# Autodesk Inventor assembly: Section 1
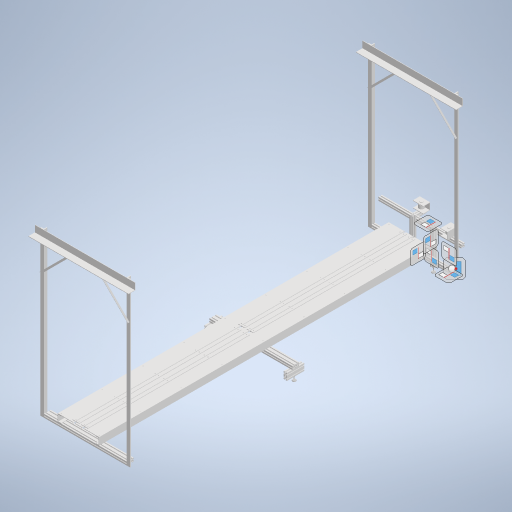
[picture p0: Inventor's stored thumbnail of the model, 512x512]
Saved by Autodesk Inventor 2023 (Build 270158030, 158C)
## iProperties
Created: 2022-06-28
Part Number: Section 1
Document SubType Name: Assembly
Designer: jeremyy
Author: jeremyy
## Documents named in this file (16)
- \\andrew.ad.cmu.edu\users\users1\jeremyy\Documents\Inventor\CMU Bridge\New folder\Section 1.iam
- \\andrew.ad.cmu.edu\users\users1\jeremyy\Documents\Inventor\CMU Bridge\New folder\LatX24in.ipt
- \\andrew.ad.cmu.edu\users\users1\jeremyy\Documents\Inventor\CMU Bridge\New folder\VertL46in.ipt
- \\andrew.ad.cmu.edu\users\users1\jeremyy\Documents\Inventor\CMU Bridge\New folder\LatL29in.ipt
- \\andrew.ad.cmu.edu\users\users1\jeremyy\Documents\Inventor\CMU Bridge\New folder\DiagL.ipt
- \\andrew.ad.cmu.edu\users\users1\jeremyy\Documents\Inventor\CMU Bridge\New folder\DiagR.ipt
- \\andrew.ad.cmu.edu\users\users1\jeremyy\Documents\Inventor\CMU Bridge\New folder\LongC96.ipt
- \\andrew.ad.cmu.edu\users\users1\jeremyy\Documents\Inventor\CMU Bridge\New folder\LatXX24in.ipt
- \\andrew.ad.cmu.edu\users\users1\jeremyy\Documents\Inventor\CMU Bridge\New folder\VertL47.25in.ipt
- \\andrew.ad.cmu.edu\users\users1\jeremyy\Documents\Inventor\CMU Bridge\New folder\LongXX5.ipt
- \\andrew.ad.cmu.edu\users\users1\jeremyy\Documents\Inventor\CMU Bridge\New folder\VertX10EndFoot.ipt
- \\andrew.ad.cmu.edu\users\users1\jeremyy\Documents\Inventor\CMU Bridge\New folder\Foot.ipt
- \\andrew.ad.cmu.edu\users\users1\jeremyy\Documents\Inventor\CMU Bridge\New folder\VertX3in.ipt
- \\andrew.ad.cmu.edu\users\users1\jeremyy\Documents\Inventor\CMU Bridge\New folder\Gear.iam
- \\andrew.ad.cmu.edu\users\users1\jeremyy\Documents\Inventor\CMU Bridge\New folder\Plate1ftx8ft.ipt
- \\andrew.ad.cmu.edu\users\users1\jeremyy\Documents\Inventor\CMU Bridge\New folder\PlateRailClamp48in.iam
## Components (32 placed, 15 different names)
1. LatX24in:1 — Mate:17, Mate:18, Flush:13, Flush:15, Mate:19, Mate:22, Flush:16, Flush:17, Mate:36, Mate:38, Flush:32, Mate:43
2. VertL46in:1 — Mate:2, Flush:5, Flush:6, Mate:4, Mate:5, Mate:21, Mate:22, Flush:16, Flush:17, Mate:45, Mate:51
3. VertL46in:2 — Mate:7, Mate:8, Mate:18, Flush:13, Flush:32
4. LatL29in:1 — Mate:2, Flush:5, Flush:6, Mate:3, Mate:6
5. DiagL:1 — Mate:3, Mate:4, Mate:5
6. DiagR:1 — Mate:6, Mate:7, Mate:8
7. LongC96:1 — Flush:12, Mate:16, Flush:14, Flush:15, Mate:20, Flush:18, Mate:23, Mate:50, Mate:51
8. LongC96:2 — Flush:12, Mate:17, Flush:14, Mate:37, Flush:34, Mate:50, Mate:52, Flush:38, Flush:39
9. LatXX24in:1 — Mate:16, Mate:19, Mate:20, Mate:21, Flush:19, Mate:33, Flush:26, Flush:27, Mate:34, Flush:28, Flush:29
10. LatXX24in:2 — Flush:18, Flush:19, Mate:23, Mate:24, Flush:20, Flush:21, Mate:25, Flush:22, Flush:23
11. VertL47.25in:1 — Mate:25, Flush:22, Flush:23, Mate:26, Flush:24, Flush:25, Mate:30, Mate:32
12. VertL47.25in:2 — Mate:24, Flush:20, Flush:21, Mate:27, Mate:29
13. LatL29in:2 — Mate:26, Flush:24, Flush:25, Mate:28, Mate:31
14. DiagR:2 — Mate:30, Mate:31, Mate:32
15. DiagL:2 — Mate:27, Mate:28, Mate:29
16. LongXX5:1 — Mate:33, Flush:26, Flush:27, Mate:41, Tangent:3, Tangent:6, Flush:47
17. LongXX5:2 — Mate:34, Flush:28, Flush:29, Mate:42, Tangent:4, Tangent:5
18. VertX10EndFoot:1 — Mate:36, Flush:31, Mate:40, Tangent:2
19. VertX10EndFoot:2 — Mate:37, Mate:38, Flush:31, Mate:39, Tangent:1, Mate:44, Mate:48, Flush:47
20. Foot:1 — Mate:39, Tangent:1
21. Foot:2 — Mate:40, Tangent:2
22. Foot:3 — Mate:41, Tangent:3, Tangent:6
23. Foot:4 — Mate:42, Tangent:4, Tangent:5
24. LatX24in:2 — Mate:43, Mate:44, Mate:45, Mate:46, Flush:33, Mate:47
25. VertX3in:1 — Mate:46, Flush:33, Flush:34, Mate:49, Flush:35, Flush:36, Flush:37
26. Gear:1 [sub-assembly] — Mate:47, Mate:48
27. Gear:2 [sub-assembly] — Mate:49, Flush:35, Flush:36, Flush:37
28. Plate1ftx8ft:1 — Mate:52, Flush:38, Flush:39, Mate:53, Flush:40, Flush:41, Mate:54, Flush:42, Flush:43, Mate:55, Mate:57
29. PlateRailClamp48in:1 [sub-assembly] — Mate:53, Flush:40, Flush:41, Mate:58, Flush:46
30. PlateRailClamp48in:2 [sub-assembly] — Mate:54, Flush:42, Flush:43, Mate:56, Flush:44, Flush:45
31. PlateRailClamp48in:3 [sub-assembly] — Mate:55, Mate:56, Flush:44, Flush:45
32. PlateRailClamp48in:4 [sub-assembly] — Mate:57, Mate:58, Flush:46
## Relationships (92: Mate 49, Flush 37, Tangent 6)
- Mate:2: VertL46in:1 ↔ LatL29in:1
- Flush:5: VertL46in:1 ↔ LatL29in:1
- Flush:6 (-38.1 mm): VertL46in:1 ↔ LatL29in:1
- Mate:3: LatL29in:1 ↔ DiagL:1
- Mate:4: VertL46in:1 ↔ DiagL:1
- Mate:5 (-266.7 mm): VertL46in:1 ↔ DiagL:1
- Mate:6: LatL29in:1 ↔ DiagR:1
- Mate:7: VertL46in:2 ↔ DiagR:1
- Mate:8 (-266.7 mm): VertL46in:2 ↔ DiagR:1
- Flush:12: LongC96:1 ↔ LongC96:2
- Mate:16: LongC96:1 ↔ LatXX24in:1
- Mate:17: LatX24in:1 ↔ LongC96:2
- Mate:18: LatX24in:1 ↔ VertL46in:2
- Flush:13: LatX24in:1 ↔ VertL46in:2
- Flush:14: LongC96:1 ↔ LongC96:2
- Flush:15: LatX24in:1 ↔ LongC96:1
- Mate:19 (-1219.2 mm): LatX24in:1 ↔ LatXX24in:1
- Mate:20: LongC96:1 ↔ LatXX24in:1
- Mate:21: VertL46in:1 ↔ LatXX24in:1
- Mate:22: LatX24in:1 ↔ VertL46in:1
- Flush:16: LatX24in:1 ↔ VertL46in:1
- Flush:17: LatX24in:1 ↔ VertL46in:1
- Flush:18: LongC96:1 ↔ LatXX24in:2
- Flush:19: LatXX24in:1 ↔ LatXX24in:2
- Mate:23: LongC96:1 ↔ LatXX24in:2
- Mate:24: LatXX24in:2 ↔ VertL47.25in:2
- Flush:20: LatXX24in:2 ↔ VertL47.25in:2
- Flush:21: LatXX24in:2 ↔ VertL47.25in:2
- Mate:25: LatXX24in:2 ↔ VertL47.25in:1
- Flush:22: LatXX24in:2 ↔ VertL47.25in:1
- Flush:23: LatXX24in:2 ↔ VertL47.25in:1
- Mate:26: VertL47.25in:1 ↔ LatL29in:2
- Flush:24: VertL47.25in:1 ↔ LatL29in:2
- Flush:25 (38.1 mm): VertL47.25in:1 ↔ LatL29in:2
- Mate:27: VertL47.25in:2 ↔ DiagL:2
- Mate:28: LatL29in:2 ↔ DiagL:2
- Mate:29 (-266.7 mm): VertL47.25in:2 ↔ DiagL:2
- Mate:30: VertL47.25in:1 ↔ DiagR:2
- Mate:31: LatL29in:2 ↔ DiagR:2
- Mate:32 (-266.7 mm): VertL47.25in:1 ↔ DiagR:2
- Mate:33: LatXX24in:1 ↔ LongXX5:1
- Flush:26: LatXX24in:1 ↔ LongXX5:1
- Flush:27 (-38.1 mm): LatXX24in:1 ↔ LongXX5:1
- Mate:34: LatXX24in:1 ↔ LongXX5:2
- Flush:28: LatXX24in:1 ↔ LongXX5:2
- Flush:29 (-38.1 mm): LatXX24in:1 ↔ LongXX5:2
- Mate:36: LatX24in:1 ↔ VertX10EndFoot:1
- Mate:37: LongC96:2 ↔ VertX10EndFoot:2
- Mate:38: LatX24in:1 ↔ VertX10EndFoot:2
- Flush:31: VertX10EndFoot:1 ↔ VertX10EndFoot:2
- Flush:32: LatX24in:1 ↔ VertL46in:2
- Mate:39: VertX10EndFoot:2 ↔ Foot:1
- Tangent:1: VertX10EndFoot:2 ↔ Foot:1
- Mate:40: VertX10EndFoot:1 ↔ Foot:2
- Tangent:2: VertX10EndFoot:1 ↔ Foot:2
- Mate:41: LongXX5:1 ↔ Foot:3
- Tangent:3 (-14.605 mm): LongXX5:1 ↔ Foot:3
- Mate:42: LongXX5:2 ↔ Foot:4
- Tangent:4 (-63.5 mm): LongXX5:2 ↔ Foot:4
- Tangent:5 (-14.605 mm): LongXX5:2 ↔ Foot:4
- Tangent:6 (-63.5 mm): LongXX5:1 ↔ Foot:3
- Mate:43 (127 mm): LatX24in:1 ↔ LatX24in:2
- Mate:44: VertX10EndFoot:2 ↔ LatX24in:2
- Mate:45: VertL46in:1 ↔ LatX24in:2
- Mate:46: LatX24in:2 ↔ VertX3in:1
- Flush:33: LatX24in:2 ↔ VertX3in:1
- Flush:34 (152.4 mm): LongC96:2 ↔ VertX3in:1
- Mate:47: LatX24in:2 ↔ Gear:1
- Mate:48 (50.8 mm): VertX10EndFoot:2 ↔ Gear:1
- Mate:49: VertX3in:1 ↔ Gear:2
- Flush:35: VertX3in:1 ↔ Gear:2
- Mate:50 (-304.8 mm): LongC96:1 ↔ LongC96:2
- Mate:51 (101.6 mm): VertL46in:1 ↔ LongC96:1
- Flush:36 (-25.4 mm): VertX3in:1 ↔ Gear:2
- Flush:37: VertX3in:1 ↔ Gear:2
- Mate:52: LongC96:2 ↔ Plate1ftx8ft:1
- Flush:38: LongC96:2 ↔ Plate1ftx8ft:1
- Flush:39: LongC96:2 ↔ Plate1ftx8ft:1
- Mate:53: Plate1ftx8ft:1 ↔ PlateRailClamp48in:1
- Flush:40: Plate1ftx8ft:1 ↔ PlateRailClamp48in:1
- Flush:41 (-95.25 mm): Plate1ftx8ft:1 ↔ PlateRailClamp48in:1
- Mate:54: Plate1ftx8ft:1 ↔ PlateRailClamp48in:2
- Flush:42: Plate1ftx8ft:1 ↔ PlateRailClamp48in:2
- Flush:43 (95.25 mm): Plate1ftx8ft:1 ↔ PlateRailClamp48in:2
- Mate:55: Plate1ftx8ft:1 ↔ PlateRailClamp48in:3
- Mate:56: PlateRailClamp48in:2 ↔ PlateRailClamp48in:3
- Flush:44: PlateRailClamp48in:2 ↔ PlateRailClamp48in:3
- Flush:45: PlateRailClamp48in:2 ↔ PlateRailClamp48in:3
- Mate:57: Plate1ftx8ft:1 ↔ PlateRailClamp48in:4
- Mate:58: PlateRailClamp48in:1 ↔ PlateRailClamp48in:4
- Flush:46: PlateRailClamp48in:1 ↔ PlateRailClamp48in:4
- Flush:47: LongXX5:1 ↔ VertX10EndFoot:2
